# Autodesk Inventor assembly: FloatingIntake
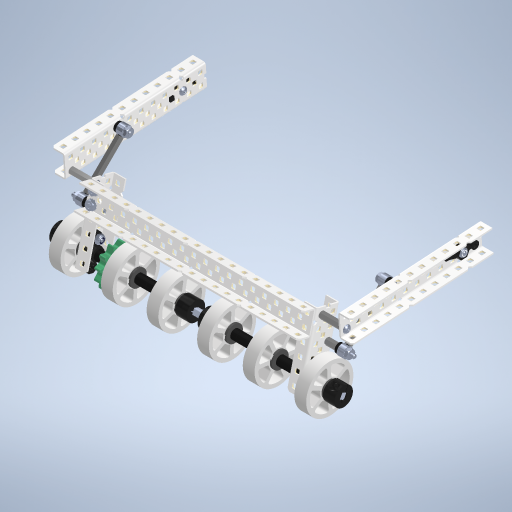
[picture p0: Inventor's stored thumbnail of the model, 512x512]
Saved by Autodesk Inventor 2023 (Build 270158000, 158)
## iProperties
Created: 2022-09-09
Part Number: FloatingIntake
Document SubType Name: Assembly
Designer: alex
Author: alex
## Documents named in this file (31)
- C:\Users\alex\Documents\GitHub\4067X_spin_up_cad\Mechanism\FloatingIntake.iam
- C:\Users\alex\Documents\GitHub\4067X_spin_up_cad\Library\Structure\C-Channels\Aluminum 1x2x1\Alu C 1x2x1x6.ipt
- C:\Users\alex\Documents\GitHub\4067X_spin_up_cad\Library\Motion\Shaft HS\Shaft HS\Shaft HS 12.0 in.ipt
- C:\Users\alex\Documents\GitHub\4067X_spin_up_cad\Library\Motion\Shaft HS\Shaft HS.ipt
- C:\Users\alex\Documents\GitHub\4067X_spin_up_cad\Library\Motion\Spacers\Spacer Nylon .375 OD\NSpacer .375 OD x .125.ipt
- C:\Users\alex\Documents\GitHub\4067X_spin_up_cad\Library\Motion\Spacers\Spacer Nylon .375 OD.ipt
- C:\Users\alex\Documents\GitHub\4067X_spin_up_cad\Library\Motion\Shaft Collar with Set Screw.ipt
- C:\Users\alex\Documents\GitHub\4067X_spin_up_cad\WithAdapter2Inch.iam
- C:\Users\alex\Documents\GitHub\4067X_spin_up_cad\Library\Structure\Standoff\Standoff 2.00.ipt
- C:\Users\alex\Documents\GitHub\4067X_spin_up_cad\Library\Structure\Standoff.ipt
- C:\Users\alex\Documents\GitHub\4067X_spin_up_cad\Library\Structure\Standoff\Standoff .50.ipt
- C:\Users\alex\Documents\GitHub\4067X_spin_up_cad\Library\Structure\Standoff\Standoff 1.00.ipt
- C:\Users\alex\Documents\GitHub\4067X_spin_up_cad\Library\Motion\Shaft HS\HS Shaft Collar.ipt
- C:\Users\alex\Documents\GitHub\4067X_spin_up_cad\Library\Structure\Hardware\Screw Steel - Star\SScrew Star Smooth 1.250.ipt
- C:\Users\alex\Documents\GitHub\4067X_spin_up_cad\Library\Structure\Hardware\Screw Steel - Star.ipt
- C:\Users\alex\Documents\GitHub\4067X_spin_up_cad\Library\Structure\Hardware\Nut Keps.ipt
- C:\Users\alex\Documents\GitHub\4067X_spin_up_cad\Library\Structure\Hardware\Screw Steel - Star\SScrew Star Smooth .290.ipt
- C:\Users\alex\Documents\GitHub\4067X_spin_up_cad\Library\Structure\Hardware\Screw Steel - Star\SScrew Star Smooth .625.ipt
- C:\Users\alex\Documents\GitHub\4067X_spin_up_cad\Library\Structure\C-Channels\Aluminum 1x2x1\Alu C 1x2x1x12.ipt
- C:\Users\alex\Documents\GitHub\4067X_spin_up_cad\Library\Motion\1-Post Bearing Flat Hex Retainer.ipt
- C:\Users\alex\Documents\GitHub\4067X_spin_up_cad\Library\Structure\Hardware\Screw Steel - Star\SScrew Star Smooth .375.ipt
- C:\Users\alex\Documents\GitHub\4067X_spin_up_cad\Library\Structure\Hardware\Nut Nylock.ipt
- C:\Users\alex\Documents\GitHub\4067X_spin_up_cad\Library\Motion\Shaft HS\HS Bearing Flat.ipt
- C:\Users\alex\Documents\GitHub\4067X_spin_up_cad\Library\Motion\Shaft HS\HS Spacer\HSpacer .0625.ipt
- C:\Users\alex\Documents\GitHub\4067X_spin_up_cad\Library\Motion\Shaft HS\HS Spacer.ipt
- C:\Users\alex\Documents\GitHub\4067X_spin_up_cad\Library\Structure\Hardware\Screw Steel - Star\SScrew Star Smooth .500.ipt
- C:\Users\alex\Documents\GitHub\4067X_spin_up_cad\Library\Structure\Hardware\Nut Thin Nylock.ipt
- C:\Users\alex\Documents\GitHub\4067X_spin_up_cad\Library\Motion\Shaft HS\HS Spacer\HSpacer .5000.ipt
- C:\Users\alex\Documents\GitHub\4067X_spin_up_cad\Library\Motion\Sprockets\HS 12T Sprocket, No Insert.ipt
- C:\Users\alex\Documents\GitHub\4067X_spin_up_cad\Library\Motion\Shaft HS\HS Spacer\HSpacer .2500.ipt
- C:\Users\alex\Documents\GitHub\4067X_spin_up_cad\Library\Structure\C-Channels\Aluminum 1x2x1\Alu C 1x2x1x19.ipt
## Components (70 placed, 25 different names)
1. Alu C 1x2x1x6:1 — Insert:63
2. Shaft HS 12.0 in:1
3. NSpacer .375 OD x .125:1
4. Shaft Collar with Set Screw:1
5. Shaft Collar with Set Screw:2
6. WithAdapter2Inch:1 [sub-assembly]
7. Standoff 2.00:1
8. Standoff .50:2
9. NSpacer .375 OD x .125:2
10. Standoff 1.00:3
11. HS Shaft Collar:1
12. SScrew Star Smooth 1.250:1
13. Nut Keps:1
14. SScrew Star Smooth .290:2
15. SScrew Star Smooth .290:3
16. SScrew Star Smooth .625:4
17. Nut Keps:2
18. Alu C 1x2x1x12:1
19. 1-Post Bearing Flat Hex Retainer:1
20. SScrew Star Smooth .375:5
21. Nut Nylock:1
22. Alu C 1x2x1x12:2
23. 1-Post Bearing Flat Hex Retainer:2
24. SScrew Star Smooth .375:6
25. Nut Nylock:2
26. SScrew Star Smooth .625:7
27. NSpacer .375 OD x .125:3
28. Shaft Collar with Set Screw:3
29. Nut Keps:3
30. SScrew Star Smooth .290:8
31. Standoff 1.00:4
32. Alu C 1x2x1x6:2
33. Shaft Collar with Set Screw:4
34. Standoff 2.00:5
35. Standoff .50:6
36. NSpacer .375 OD x .125:4
37. SScrew Star Smooth 1.250:9
38. Nut Keps:4
39. HS Bearing Flat:1
40. HSpacer .0625:1
41. SScrew Star Smooth .500:10
42. Nut Thin Nylock:1
43. HSpacer .0625:2
44. WithAdapter2Inch:2 [sub-assembly]
45. HS Shaft Collar:2
46. HS Bearing Flat:2
47. Nut Thin Nylock:2
48. SScrew Star Smooth .500:11
49. WithAdapter2Inch:3 [sub-assembly]
50. HSpacer .5000:3
51. HSpacer .5000:4
52. WithAdapter2Inch:4 [sub-assembly]
53. WithAdapter2Inch:5 [sub-assembly]
54. HSpacer .5000:5
55. HSpacer .5000:6
56. WithAdapter2Inch:6 [sub-assembly]
57. HSpacer .5000:7
58. HSpacer .5000:8
59. HS 12T Sprocket, No Insert:1
60. HSpacer .5000:9
61. HSpacer .2500:10
62. HSpacer .2500:11
63. HS Shaft Collar:3
64. HS Shaft Collar:4
65. Alu C 1x2x1x19:1 — Insert:63
66. SScrew Star Smooth .290:12
67. SScrew Star Smooth .290:13
68. SScrew Star Smooth .290:14
69. Nut Keps:5
70. Nut Keps:6
## Relationships (90: Insert 63, Mate 24, Flush 3)
- [Mate]: Alu C 1x2x1x6:1 ↔ Shaft HS 12.0 in:1
- [Insert]: NSpacer .375 OD x .125:1 ↔ Shaft Collar with Set Screw:1
- [Mate]: Alu C 1x2x1x6:1 ↔ Shaft Collar with Set Screw:2
- [Mate]: Shaft Collar with Set Screw:1 ↔ Shaft Collar with Set Screw:2
- [Mate]: Shaft HS 12.0 in:1 ↔ WithAdapter2Inch:1
- [Mate]: Shaft HS 12.0 in:1 ↔ WithAdapter2Inch:1
- [Insert] (-0.3556 mm): Shaft Collar with Set Screw:2 ↔ Standoff 2.00:1
- [Mate] (-0.3556 mm): Shaft Collar with Set Screw:1 ↔ Standoff 2.00:1
- [Insert]: Standoff .50:2 ↔ NSpacer .375 OD x .125:2
- [Insert]: Alu C 1x2x1x6:1 ↔ Standoff .50:2
- [Insert]: Alu C 1x2x1x6:1 ↔ Standoff 1.00:3
- [Mate]: WithAdapter2Inch:1 ↔ HS Shaft Collar:1
- [Mate]: Shaft HS 12.0 in:1 ↔ HS Shaft Collar:1
- [Mate]: Shaft HS 12.0 in:1 ↔ HS Shaft Collar:1
- [Flush] (1.27 mm): Shaft HS 12.0 in:1 ↔ HS Shaft Collar:1
- [Insert]: Alu C 1x2x1x6:1 ↔ SScrew Star Smooth 1.250:1
- [Insert]: Shaft Collar with Set Screw:2 ↔ Nut Keps:1
- [Insert]: Alu C 1x2x1x6:1 ↔ SScrew Star Smooth .290:2
- [Insert]: Shaft Collar with Set Screw:1 ↔ Nut Keps:2
- [Insert]: Standoff 1.00:3 ↔ Alu C 1x2x1x12:1
- [Insert]: SScrew Star Smooth .290:3 ↔ Alu C 1x2x1x12:1
- [Insert]: NSpacer .375 OD x .125:1 ↔ Alu C 1x2x1x12:1
- [Insert]: SScrew Star Smooth .625:4 ↔ Alu C 1x2x1x12:1
- [Insert]: Alu C 1x2x1x12:1 ↔ 1-Post Bearing Flat Hex Retainer:1
- [Mate]: Alu C 1x2x1x12:1 ↔ 1-Post Bearing Flat Hex Retainer:1
- [Insert]: Alu C 1x2x1x12:1 ↔ SScrew Star Smooth .375:5
- [Insert]: 1-Post Bearing Flat Hex Retainer:1 ↔ Nut Nylock:1
- [Insert]: Alu C 1x2x1x12:2 ↔ 1-Post Bearing Flat Hex Retainer:2
- [Mate]: Alu C 1x2x1x12:2 ↔ 1-Post Bearing Flat Hex Retainer:2
- [Insert]: Alu C 1x2x1x12:2 ↔ SScrew Star Smooth .375:6
- [Insert]: 1-Post Bearing Flat Hex Retainer:2 ↔ Nut Nylock:2
- [Insert]: Alu C 1x2x1x12:2 ↔ SScrew Star Smooth .625:7
- [Insert]: NSpacer .375 OD x .125:3 ↔ Shaft Collar with Set Screw:3
- [Insert]: Shaft Collar with Set Screw:3 ↔ Nut Keps:3
- [Insert]: Alu C 1x2x1x12:2 ↔ NSpacer .375 OD x .125:3
- [Flush]: Alu C 1x2x1x12:1 ↔ Alu C 1x2x1x12:2
- [Insert]: Alu C 1x2x1x12:2 ↔ SScrew Star Smooth .290:8
- [Insert]: Alu C 1x2x1x12:2 ↔ Standoff 1.00:4
- [Insert]: Standoff 1.00:4 ↔ Alu C 1x2x1x6:2
- [Insert] (-0.3556 mm): Shaft Collar with Set Screw:4 ↔ Standoff 2.00:5
- [Insert] (-0.3556 mm): Shaft Collar with Set Screw:3 ↔ Standoff 2.00:5
- [Mate]: Alu C 1x2x1x6:2 ↔ Shaft Collar with Set Screw:4
- [Insert]: Standoff .50:6 ↔ NSpacer .375 OD x .125:4
- [Insert]: Alu C 1x2x1x6:2 ↔ Standoff .50:6
- [Insert]: Alu C 1x2x1x6:2 ↔ SScrew Star Smooth 1.250:9
- [Insert]: Shaft Collar with Set Screw:4 ↔ Nut Keps:4
- [Insert]: Alu C 1x2x1x6:1 ↔ HS Bearing Flat:1
- [Mate]: Alu C 1x2x1x6:1 ↔ HS Bearing Flat:1
- [Mate]: Shaft HS 12.0 in:1 ↔ HSpacer .0625:1
- [Mate]: Alu C 1x2x1x6:1 ↔ HSpacer .0625:1
- [Mate]: WithAdapter2Inch:1 ↔ HSpacer .0625:1
- [Insert]: Alu C 1x2x1x6:1 ↔ SScrew Star Smooth .500:10
- [Insert]: HS Bearing Flat:1 ↔ Nut Thin Nylock:1
- [Mate]: Shaft HS 12.0 in:1 ↔ HSpacer .0625:2
- [Mate]: Alu C 1x2x1x6:2 ↔ HSpacer .0625:2
- [Mate]: Shaft HS 12.0 in:1 ↔ WithAdapter2Inch:2
- [Mate]: Shaft HS 12.0 in:1 ↔ WithAdapter2Inch:2
- [Mate]: HSpacer .0625:2 ↔ WithAdapter2Inch:2
- [Mate]: Shaft HS 12.0 in:1 ↔ HS Shaft Collar:2
- [Mate]: Shaft HS 12.0 in:1 ↔ HS Shaft Collar:2
- [Mate]: WithAdapter2Inch:2 ↔ HS Shaft Collar:2
- [Insert]: HS Bearing Flat:2 ↔ Nut Thin Nylock:2
- [Insert]: Alu C 1x2x1x6:2 ↔ HS Bearing Flat:2
- [Insert]: Alu C 1x2x1x6:2 ↔ HS Bearing Flat:2
- [Insert]: Alu C 1x2x1x6:2 ↔ SScrew Star Smooth .500:11
- [Insert]: WithAdapter2Inch:3 ↔ HSpacer .5000:3
- [Insert]: HSpacer .5000:5 ↔ HSpacer .5000:6
- [Insert]: HSpacer .5000:7 ↔ HSpacer .5000:8
- [Insert]: WithAdapter2Inch:6 ↔ HSpacer .5000:7
- [Insert]: HSpacer .5000:6 ↔ WithAdapter2Inch:6
- [Insert]: HS Bearing Flat:1 ↔ HSpacer .5000:8
- [Insert]: HS Bearing Flat:2 ↔ HSpacer .5000:9
- [Insert]: HS 12T Sprocket, No Insert:1 ↔ HSpacer .5000:9
- [Insert]: WithAdapter2Inch:3 ↔ HS 12T Sprocket, No Insert:1
- [Insert]: HSpacer .5000:3 ↔ HSpacer .5000:4
- [Insert]: HSpacer .5000:4 ↔ HSpacer .2500:10
- [Insert]: WithAdapter2Inch:4 ↔ HSpacer .2500:10
- [Insert]: HSpacer .5000:5 ↔ HSpacer .2500:11
- [Insert]: WithAdapter2Inch:5 ↔ HSpacer .2500:11
- [Insert]: WithAdapter2Inch:4 ↔ HS Shaft Collar:3
- [Insert]: WithAdapter2Inch:5 ↔ HS Shaft Collar:4
- [Insert]: Alu C 1x2x1x6:2 ↔ Alu C 1x2x1x19:1
- [Insert]: Alu C 1x2x1x6:2 ↔ Alu C 1x2x1x19:1
- [Flush]: Alu C 1x2x1x6:1 ↔ Alu C 1x2x1x6:2
- [Insert]: Alu C 1x2x1x6:2 ↔ SScrew Star Smooth .290:12
- [Insert]: Alu C 1x2x1x6:2 ↔ SScrew Star Smooth .290:13
- [Insert]: Alu C 1x2x1x6:2 ↔ SScrew Star Smooth .290:14
- [Insert]: Alu C 1x2x1x19:1 ↔ Nut Keps:5
- [Insert]: Alu C 1x2x1x19:1 ↔ Nut Keps:6
- Insert:63: Alu C 1x2x1x6:1 ↔ Alu C 1x2x1x19:1
## Named parameters: d253_d244 = 0 mm, d265_d262_d260_d258 = 0 mm, d268_d262_d260_d258 = 0 mm, d269_d263_d261 = 0 mm, d224_d43 = 0 mm, d225_d78 = 0 mm, d231_d48 = -0.3556 mm, d234_d52 = 0 mm, d205_d144 = 0 mm, d206_d145 = 0 mm, d207_d146 = 0 mm, d208_d147 = 0 mm
